# Autodesk Inventor assembly: 0_Entire_Assembly
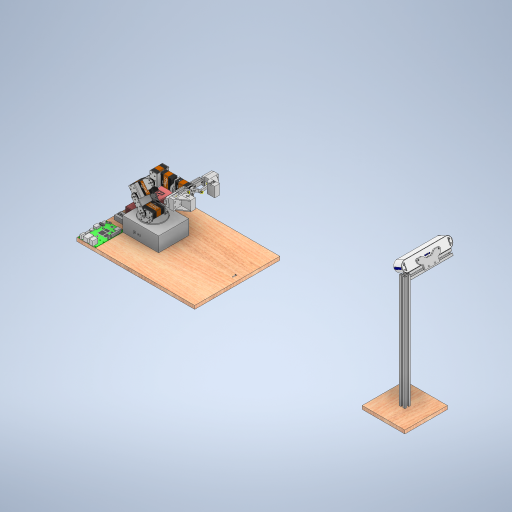
[picture p0: Inventor's stored thumbnail of the model, 512x512]
Saved by Autodesk Inventor 2024.2 (Build 282272000, 272)
## iProperties
Created: 2023-08-24
Part Number: 0_Entire_Assembly
Document SubType Name: Assembly
Designer: chanh
Author: chanh
## Documents named in this file (5)
- C:\Users\박동준\OneDrive - 연세대학교 (Yonsei University)\바탕 화면\박동준\대학생할\로봇\Humanoid\7축 매니퓰레이터\하드웨어\rh_plus_7_axis_robot_arm_hardware\Assembly\0_Entire_Assembly.iam
- C:\Users\박동준\OneDrive - 연세대학교 (Yonsei University)\바탕 화면\박동준\대학생할\로봇\Humanoid\7축 매니퓰레이터\하드웨어\rh_plus_7_axis_robot_arm_hardware\Assembly\2_Arm.iam
- C:\Users\박동준\OneDrive - 연세대학교 (Yonsei University)\바탕 화면\박동준\대학생할\로봇\Humanoid\7축 매니퓰레이터\하드웨어\rh_plus_7_axis_robot_arm_hardware\Assembly\3_Gripper.iam
- C:\Users\박동준\OneDrive - 연세대학교 (Yonsei University)\바탕 화면\박동준\대학생할\로봇\Humanoid\7축 매니퓰레이터\하드웨어\rh_plus_7_axis_robot_arm_hardware\Assembly\1_Base.iam
- C:\Users\박동준\OneDrive - 연세대학교 (Yonsei University)\바탕 화면\박동준\대학생할\로봇\Humanoid\7축 매니퓰레이터\하드웨어\rh_plus_7_axis_robot_arm_hardware\Assembly\4_Camera.iam
## Components (4 placed, 4 different names)
1. 1_Base:1 [sub-assembly] — Flush:4, Flush:5, Flush:6, Flush:7, Mate:1
2. 2_Arm:1 [sub-assembly] — Flush:1, Flush:2, Flush:3, Rigid:1, Flush:4, Flush:5, Flush:6, Mate:2
3. 3_Gripper:1 [sub-assembly] — Rigid:1
4. 4_Camera:1 [sub-assembly] — Flush:7, Mate:1, Mate:2
## Relationships (10: Flush 7, Mate 2, WeldJoint 1)
- Flush:1: 2_Arm:1
- Flush:2: 2_Arm:1
- Flush:3: 2_Arm:1
- Rigid:1 [WeldJoint]: 2_Arm:1 ↔ 3_Gripper:1
- Flush:4: 1_Base:1 ↔ 2_Arm:1
- Flush:5: 1_Base:1 ↔ 2_Arm:1
- Flush:6: 1_Base:1 ↔ 2_Arm:1
- Flush:7: 1_Base:1 ↔ 4_Camera:1
- Mate:1 (600 mm): 1_Base:1 ↔ 4_Camera:1
- Mate:2: 2_Arm:1 ↔ 4_Camera:1
